# Autodesk Inventor assembly: Montagem
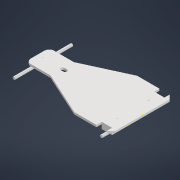
[picture p0: Inventor's stored thumbnail of the model, 180x180]
Saved by Autodesk Inventor 2022 (Build 260153000, 153)
## iProperties
Created: 2022-06-09
Part Number: Montagem
Document SubType Name: Assembly
Designer: Gugarauj07
Author: Gugarauj07
## Documents named in this file (4)
- C:\Users\Gugarauj07\PycharmProjects\Eletronica_2022\CADS\Carrinho_Rolima\Montagem\Montagem.iam
- C:\Users\Gugarauj07\PycharmProjects\Eletronica_2022\CADS\Carrinho_Rolima\Base.ipt
- C:\Users\Gugarauj07\PycharmProjects\Eletronica_2022\CADS\Carrinho_Rolima\Eixo_dianteiro.ipt
- C:\Users\Gugarauj07\PycharmProjects\Eletronica_2022\CADS\Carrinho_Rolima\Eixo_traseiro.ipt
## Components (3 placed, 3 different names)
1. Base:1 — Mate:1, Mate:2, Mate:3
2. Eixo_dianteiro:1 — Mate:1
3. Eixo_traseiro:1 — Mate:2, Mate:3
## Relationships (3: Mate 3)
- Mate:1: Base:1 ↔ Eixo_dianteiro:1
- Mate:2: Base:1 ↔ Eixo_traseiro:1
- Mate:3: Base:1 ↔ Eixo_traseiro:1
